# Autodesk Inventor assembly: Center Wheel
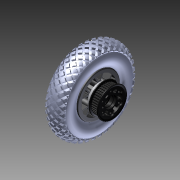
[picture p0: Inventor's stored thumbnail of the model, 180x180]
Saved by Autodesk Inventor 2014 SP1 (Build 180222100, 222)
## iProperties
Created: 2014-01-21
Part Number: Center Wheel
Document SubType Name: Assembly
Designer: Nick
Author: Nick
## Documents named in this file (5)
- D:\Dropbox\School\PurdueFIRST\PFP Robot\PFP Robot with Cart\Center Wheel.iam
- D:\Dropbox\School\PurdueFIRST\PFP Robot\PFP Robot with Cart\PneumaticWheel_am-0970.iam
- D:\Dropbox\School\PurdueFIRST\PFP Robot\PFP Robot with Cart\Pulley.iam
- D:\Dropbox\School\PurdueFIRST\PFP Robot\PFP Robot with Cart\Imported Components\500_hex_hub\500_hex_hub.ipt
- D:\Dropbox\School\PurdueFIRST\PFP Robot\PFP Robot with Cart\Rough_Spacer.ipt
## Components (7 placed, 4 different names)
1. PneumaticWheel_am-0970:1 [sub-assembly] — Mate:7, Mate:13, Mate:16, Mate:17, Mate:20
2. Pulley:1 [sub-assembly] — Mate:5, Mate:6, Mate:11, Mate:22
3. Pulley:2 [sub-assembly] — Mate:1, Mate:3, Mate:15, Mate:19
4. 500_hex_hub:1 — Mate:1, Mate:3, Mate:17, Mate:18
5. 500_hex_hub:2 — Mate:5, Mate:6, Mate:20, Mate:21
6. Rough_Spacer:1 — Mate:7, Mate:15, Mate:16, Mate:18, Mate:19
7. Rough_Spacer:2 — Mate:11, Mate:13, Mate:21, Mate:22
## Relationships (15: Mate 15)
- Mate:1: Pulley:2 ↔ 500_hex_hub:1
- Mate:3: Pulley:2 ↔ 500_hex_hub:1
- Mate:5: Pulley:1 ↔ 500_hex_hub:2
- Mate:6: Pulley:1 ↔ 500_hex_hub:2
- Mate:7: PneumaticWheel_am-0970:1 ↔ Rough_Spacer:1
- Mate:11: Pulley:1 ↔ Rough_Spacer:2
- Mate:13: PneumaticWheel_am-0970:1 ↔ Rough_Spacer:2
- Mate:15: Pulley:2 ↔ Rough_Spacer:1
- Mate:16: PneumaticWheel_am-0970:1 ↔ Rough_Spacer:1
- Mate:17: PneumaticWheel_am-0970:1 ↔ 500_hex_hub:1
- Mate:18: 500_hex_hub:1 ↔ Rough_Spacer:1
- Mate:19: Pulley:2 ↔ Rough_Spacer:1
- Mate:20: PneumaticWheel_am-0970:1 ↔ 500_hex_hub:2
- Mate:21: 500_hex_hub:2 ↔ Rough_Spacer:2
- Mate:22: Pulley:1 ↔ Rough_Spacer:2
